# Autodesk Inventor assembly: Main
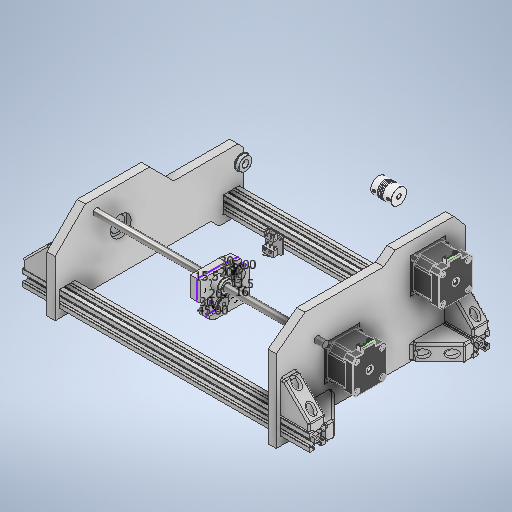
[picture p0: Inventor's stored thumbnail of the model, 512x512]
Saved by Autodesk Inventor 2025.3 (Build 293356030, 356C)
## iProperties
Created: 2025-09-01
Part Number: Main
Document SubType Name: Assembly
Designer: tvoko
Author: tvoko
## iProperties of the stored document 3.Linear Bearing-LM8UU.ipt
Created: 2022-04-19
Part Number: 3.Linear Bearing-LM8UU
Material: Generic
Description: STEP AP203
Document SubType Name: Modeling
Designer: tvoko
Density: 1 g/cm^3
Appearance: Default
Sending System: SolidWorks 2017
Preprocessor: SwSTEP 2.0
Title: 3.Linear Bearing-LM8UU.STEP
Revision Number: ANY
## Documents named in this file (15)
- C:\Users\tvoko\Github\DIY-Coil-Winder\CAD\Main.iam
- C:\Users\tvoko\Github\DIY-Coil-Winder\CAD\2020-Profile.ipt
- C:\Users\tvoko\Github\DIY-Coil-Winder\CAD\Motor-Side.ipt
- C:\Users\tvoko\Github\DIY-Coil-Winder\CAD\Imports\NEMA 17 Stepper Motor 39mm-NEMA 17 Stepper Motor 39mm\barre T8 v1\barre T8 v1.ipt
- C:\Users\tvoko\Github\DIY-Coil-Winder\CAD\Imports\NEMA 17 Stepper Motor 39mm-NEMA 17 Stepper Motor 39mm\Creality Limit Switch\Creality Limit Switch.ipt
- C:\Users\tvoko\Github\DIY-Coil-Winder\CAD\Imports\NEMA 17 Stepper Motor 39mm-NEMA 17 Stepper Motor 39mm\F688ZZ Miniature Flanged Ball Bearing Low Detail\F688ZZ Miniature Flanged Ball Bearing Low Detail.ipt
- C:\Users\tvoko\Github\DIY-Coil-Winder\CAD\Imports\NEMA 17 Stepper Motor 39mm-NEMA 17 Stepper Motor 39mm\Flexible_Shaft_Coupling_5_to_8mm v7\Flexible_Shaft_Coupling_5_to_8mm v7.ipt
- C:\Users\tvoko\Github\DIY-Coil-Winder\CAD\Imports\NEMA 17 Stepper Motor 39mm-NEMA 17 Stepper Motor 39mm\NEMA 17 Stepper Motor 39mm-NEMA 17 Stepper Motor 39mm\NEMA 17 Stepper Motor 39mm-NEMA 17 Stepper Motor 39m.ipt
- C:\Users\tvoko\Github\DIY-Coil-Winder\CAD\Imports\NEMA 17 Stepper Motor 39mm-NEMA 17 Stepper Motor 39mm\T8 Nut 1.5\T8 Nut 1.5.ipt
- C:\Users\tvoko\Github\DIY-Coil-Winder\CAD\Imports\M8x400-StainlessSteelRod.ipt
- **C:\Users\tvoko\Github\DIY-Coil-Winder\CAD\Main.iam*LocalDocs*xAaaaqkbaAaaaaaaaAaaaakp3Be*3.Linear Bearing-LM8UU.ipt
- C:\Users\tvoko\Github\DIY-Coil-Winder\CAD\Imports\uxcell_V624ZZ_4mmx13mmx6mm.ipt
- C:\Users\tvoko\Github\DIY-Coil-Winder\CAD\GuideBlock.ipt
- C:\Users\tvoko\Github\DIY-Coil-Winder\CAD\Brace-Side.ipt
- C:\Users\tvoko\Github\DIY-Coil-Winder\CAD\Imports\3.Linear Bearing-LM8UU.STEP
## Components (18 placed, 13 different names)
1. 2020-Profile:1 — Mate:7, Mate:8, Mate:9, Mate:13
2. Motor-Side:1 — Mate:12, Mate:13, Mate:14, Mate:15, Mate:16, Mate:17, Mate:18, Mate:19, Mate:20, Flush:1, Flush:2, Flush:3, Flush:5
3. 2020-Profile:2 — Mate:10, Mate:11, Mate:12, Flush:1, Flush:4
4. barre T8 v1:1 — Mate:35, Mate:36, Mate:37, Mate:38
5. Creality Limit Switch:1
6. F688ZZ Miniature Flanged Ball Bearing Low Detail:1 — Mate:38, Mate:39
7. Flexible_Shaft_Coupling_5_to_8mm v7:1 — Mate:2, Mate:3, Mate:35, Mate:36
8. NEMA 17 Stepper Motor 39mm-NEMA 17 Stepper Motor 39m:1 — Mate:2, Mate:3, Mate:14, Mate:15, Mate:16
9. T8 Nut 1.5:1 — Mate:27, Mate:28, Mate:29, Mate:37
10. NEMA 17 Stepper Motor 39mm-NEMA 17 Stepper Motor 39m:2 — Mate:17, Mate:18, Mate:19
11. Flexible_Shaft_Coupling_5_to_8mm v7:2
12. F688ZZ Miniature Flanged Ball Bearing Low Detail:2
13. M8x400-StainlessSteelRod:1 — Mate:20, Mate:22, Flush:5
14. 3.Linear Bearing-LM8UU:1 — Mate:22, Mate:26, Mate:30
15. uxcell_V624ZZ_4mmx13mmx6mm:1 — Mate:31, Mate:34
16. uxcell_V624ZZ_4mmx13mmx6mm:2 — Mate:32, Mate:33
17. GuideBlock:1 — Mate:26, Mate:27, Mate:28, Mate:29, Mate:30, Mate:31, Mate:32, Mate:33, Mate:34
18. Brace-Side:1 — Flush:2, Flush:3, Flush:4, Mate:39
## Relationships (36: Mate 31, Flush 5)
- Mate:2: Flexible_Shaft_Coupling_5_to_8mm v7:1 ↔ NEMA 17 Stepper Motor 39mm-NEMA 17 Stepper Motor 39m:1
- Mate:3: Flexible_Shaft_Coupling_5_to_8mm v7:1 ↔ NEMA 17 Stepper Motor 39mm-NEMA 17 Stepper Motor 39m:1
- Mate:7: 2020-Profile:1
- Mate:8: 2020-Profile:1
- Mate:9: 2020-Profile:1
- Mate:10: 2020-Profile:2
- Mate:11: 2020-Profile:2
- Mate:12: Motor-Side:1 ↔ 2020-Profile:2
- Mate:13: 2020-Profile:1 ↔ Motor-Side:1
- Mate:14: Motor-Side:1 ↔ NEMA 17 Stepper Motor 39mm-NEMA 17 Stepper Motor 39m:1
- Mate:15: Motor-Side:1 ↔ NEMA 17 Stepper Motor 39mm-NEMA 17 Stepper Motor 39m:1
- Mate:16: Motor-Side:1 ↔ NEMA 17 Stepper Motor 39mm-NEMA 17 Stepper Motor 39m:1
- Mate:17: Motor-Side:1 ↔ NEMA 17 Stepper Motor 39mm-NEMA 17 Stepper Motor 39m:2
- Mate:18: Motor-Side:1 ↔ NEMA 17 Stepper Motor 39mm-NEMA 17 Stepper Motor 39m:2
- Mate:19: Motor-Side:1 ↔ NEMA 17 Stepper Motor 39mm-NEMA 17 Stepper Motor 39m:2
- Mate:20: Motor-Side:1 ↔ M8x400-StainlessSteelRod:1
- Mate:22: M8x400-StainlessSteelRod:1 ↔ 3.Linear Bearing-LM8UU:1
- Mate:26: 3.Linear Bearing-LM8UU:1 ↔ GuideBlock:1
- Mate:27: T8 Nut 1.5:1 ↔ GuideBlock:1
- Mate:28: T8 Nut 1.5:1 ↔ GuideBlock:1
- Mate:29: T8 Nut 1.5:1 ↔ GuideBlock:1
- Mate:30: 3.Linear Bearing-LM8UU:1 ↔ GuideBlock:1
- Mate:31: uxcell_V624ZZ_4mmx13mmx6mm:1 ↔ GuideBlock:1
- Mate:32: uxcell_V624ZZ_4mmx13mmx6mm:2 ↔ GuideBlock:1
- Mate:33: uxcell_V624ZZ_4mmx13mmx6mm:2 ↔ GuideBlock:1
- Mate:34: uxcell_V624ZZ_4mmx13mmx6mm:1 ↔ GuideBlock:1
- Mate:35: barre T8 v1:1 ↔ Flexible_Shaft_Coupling_5_to_8mm v7:1
- Mate:36: barre T8 v1:1 ↔ Flexible_Shaft_Coupling_5_to_8mm v7:1
- Mate:37: barre T8 v1:1 ↔ T8 Nut 1.5:1
- Flush:1: Motor-Side:1 ↔ 2020-Profile:2
- Flush:2: Motor-Side:1 ↔ Brace-Side:1
- Flush:3: Motor-Side:1 ↔ Brace-Side:1
- Mate:38: barre T8 v1:1 ↔ F688ZZ Miniature Flanged Ball Bearing Low Detail:1
- Flush:4: 2020-Profile:2 ↔ Brace-Side:1
- Flush:5 (-10 mm): Motor-Side:1 ↔ M8x400-StainlessSteelRod:1
- Mate:39: F688ZZ Miniature Flanged Ball Bearing Low Detail:1 ↔ Brace-Side:1
